# Autodesk Inventor assembly: VTC1
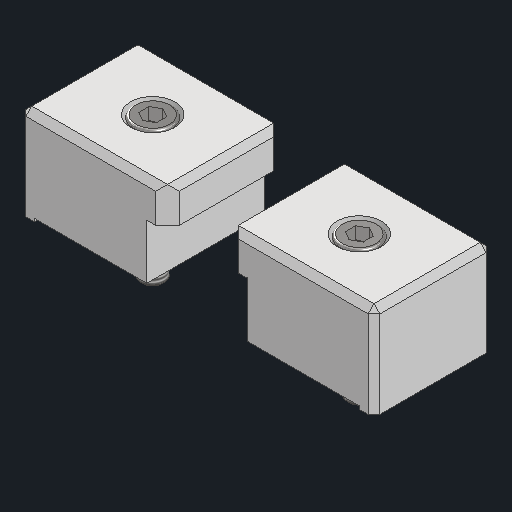
[picture p0: Inventor's stored thumbnail of the model, 512x512]
Saved by Autodesk Inventor 2024.3 (Build 283343000, 343)
## iProperties
Created: 2024-02-28
Part Number: VTC1
Document SubType Name: Assembly
Designer: fablabadmin
Author: fablabadmin
## Documents named in this file (3)
- C:\Users\fablabadmin\Documents\_Benjamin_S\_3dCAD\HHVerkstad\ViseToeClamp\VTC1.iam
- C:\Users\fablabadmin\Documents\_Benjamin_S\_3dCAD\HHVerkstad\ViseToeClamp\VTC1-001.ipt
- C:\Users\fablabadmin\Documents\Inventor\Content Center Files\R2024\en-US\AS 1420\AS 1420 - 1973 - M8 x 40.ipt
## Components (4 placed, 2 different names)
1. VTC1-001:1 — Flush:1, Flush:2, Mate:1, Symmetry:1, Symmetry:2, Insert:2
2. VTC1-001:2 — Flush:1, Flush:2, Mate:1, Symmetry:1, Flush:3, Symmetry:2, Insert:1
3. AS 1420 - Metric M8 x 40:1 — Insert:1
4. AS 1420 - Metric M8 x 40:2 — Insert:2
## Relationships (8: Flush 3, Symmetry 2, Insert 2, Mate 1)
- Flush:1: VTC1-001:1 ↔ VTC1-001:2
- Flush:2: VTC1-001:1 ↔ VTC1-001:2
- Mate:1 (20 mm): VTC1-001:1 ↔ VTC1-001:2
- Symmetry:1: VTC1-001:1 ↔ VTC1-001:2
- Flush:3: VTC1-001:2
- Symmetry:2: VTC1-001:1 ↔ VTC1-001:2
- Insert:1: VTC1-001:2 ↔ AS 1420 - Metric M8 x 40:1
- Insert:2: VTC1-001:1 ↔ AS 1420 - Metric M8 x 40:2
